# Autodesk Inventor assembly: Placed corner cabinet door
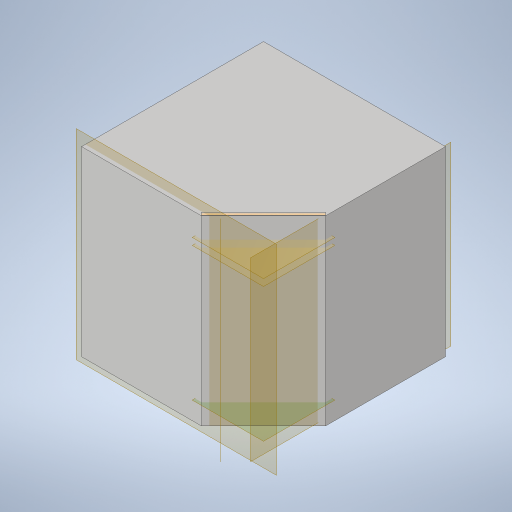
[picture p0: Inventor's stored thumbnail of the model, 512x512]
Saved by Autodesk Inventor 2024 (Build 280153000, 153)
## iProperties
RuleStatus: InUse
Created: 2017-01-20
Part Number: Placed corner cabinet door
Document SubType Name: Assembly
Designer: SvetlanaB
Author: SvetlanaB
## Documents named in this file (6)
- C:\W4INV 2024 Design\iBOX LIBRARY\Kitchen\Doors\Corner cabinet door 135 degrees hinges\corner cabinet door.iam
- C:\W4INV 2024 Design\iBOX LIBRARY\Kitchen\Doors\Corner cabinet door 135 degrees hinges\Skeleton.ipt
- C:\W4INV 2024 Design\iBOX LIBRARY\Kitchen\Doors\Corner cabinet door 135 degrees hinges\Door.ipt
- C:\W4INV 2024 Design\_LIBRARY\Hinges\45 DEGREE HINGE\45 Degree Hinge with Wood Screws And Cup Fixing Wood Screws.iam
- C:\W4INV 2024 Design\iBOX LIBRARY\Kitchen\Doors\Corner cabinet door 135 degrees hinges\corner cabinet door concept.ipt
- C:\W4INV 2023 Design\LIBRARY\Hinges\45 DEGREE HINGE.iam
## Components (5 placed, 3 different names)
1. @Skeleton:1 — Flush:11, Flush:12
2. Door:1 — Flush:1, Flush:2, Mate:10, Mate:11, Flush:9, Flush:10
3. 45 Degree Hinge with Wood Screws And Cup Fixing Wood Screws:1 [sub-assembly] — Mate:10, Right top hinge, Mate:13, Left top hinge
4. 45 Degree Hinge with Wood Screws And Cup Fixing Wood Screws:2 [sub-assembly] — Mate:11, Right bottom hinge, Mate:12, Left bottom hinge
5. @Skeleton
## Relationships (14: Flush 10, Mate 4)
- Flush:1 (-64 mm): Door:1
- Flush:2 (-128 mm): Door:1
- Mate:10: Door:1 ↔ 45 Degree Hinge with Wood Screws And Cup Fixing Wood Screws:1
- Right top hinge [Flush]: 45 Degree Hinge with Wood Screws And Cup Fixing Wood Screws:1
- Mate:11: Door:1 ↔ 45 Degree Hinge with Wood Screws And Cup Fixing Wood Screws:2
- Right bottom hinge [Flush]: 45 Degree Hinge with Wood Screws And Cup Fixing Wood Screws:2
- Flush:9 (-96 mm): Door:1
- Flush:10 (-96 mm): Door:1
- Mate:12: 45 Degree Hinge with Wood Screws And Cup Fixing Wood Screws:2
- Mate:13: 45 Degree Hinge with Wood Screws And Cup Fixing Wood Screws:1
- Flush:11 (-18 mm): @Skeleton:1
- Flush:12 (-18 mm): @Skeleton:1
- Left top hinge [Flush]: 45 Degree Hinge with Wood Screws And Cup Fixing Wood Screws:1
- Left bottom hinge [Flush]: 45 Degree Hinge with Wood Screws And Cup Fixing Wood Screws:2
## Named parameters: Panel_thickness = 18 mm, Side_allowance = 3 mm
